# Autodesk Inventor assembly: Montagem1
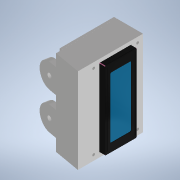
[picture p0: Inventor's stored thumbnail of the model, 180x180]
Saved by Autodesk Inventor 2022 (Build 260153000, 153)
## iProperties
Created: 2022-03-11
Part Number: Montagem1
Document SubType Name: Assembly
Designer: Guilherme
Author: Guilherme
## Documents named in this file (4)
- G:\Meu Drive\Projetos\Projeto 2020 2021\Eletrônica 2020-2021\Projeção mecânica\caixa display\Montagem1.iam
- G:\Meu Drive\Projetos\Projeto 2020 2021\Eletrônica 2020-2021\Projeção mecânica\caixa display\caica display.ipt
- G:\Meu Drive\Projetos\Projeto 2020 2021\Eletrônica 2020-2021\Projeção mecânica\caixa display\lcd 20x4.ipt
- G:\Meu Drive\Projetos\Projeto 2020 2021\Eletrônica 2020-2021\Projeção mecânica\caixa display\tampa.ipt
## Components (3 placed, 3 different names)
1. caica display:1 — Coincidente:1, Coincidente:2, Alinhado:1, Alinhado:2, Alinhado:3, Coincidente:3, Coincidente:4
2. lcd 20x4:1 — Coincidente:1, Coincidente:2
3. tampa:1 — Alinhado:1, Alinhado:2, Alinhado:3, Coincidente:3, Coincidente:4
## Relationships (7: Mate 4, Flush 3)
- Coincidente:1 [Mate]: caica display:1 ↔ lcd 20x4:1
- Coincidente:2 [Mate]: caica display:1 ↔ lcd 20x4:1
- Alinhado:1 [Flush]: caica display:1 ↔ tampa:1
- Alinhado:2 [Flush]: caica display:1 ↔ tampa:1
- Alinhado:3 [Flush]: caica display:1 ↔ tampa:1
- Coincidente:3 [Mate]: caica display:1 ↔ tampa:1
- Coincidente:4 [Mate]: caica display:1 ↔ tampa:1
